# Autodesk Inventor assembly: 14inLift
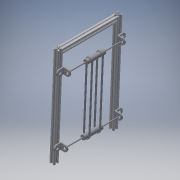
[picture p0: Inventor's stored thumbnail of the model, 180x180]
Saved by Autodesk Inventor 2016 (Build 200138000, 138)
## iProperties
Created: 2016-12-21
Part Number: 14inLift
Document SubType Name: Assembly
Designer: RoboticsUser
Author: RoboticsUser
## Documents named in this file (5)
- C:\Robotics\CAD\2016-17_CAD\12inLift (2).iam
- C:\Robotics\CAD\COTSParts\Bosch Extrusion\Bosch 20x20 16.66 -.ipt
- C:\Robotics\CAD\COTSParts\Actobotics\545 parts\545400_MIR.ipt
- C:\Robotics\CAD\COTSParts\Bosch Extrusion\Bosch 20x20 9 in actual.ipt
- C:\Robotics\CAD\2016-17_CAD\12inlift.iam
## Components (8 placed, 4 different names)
1. Bosch 20x20 16.66 -:1 — Mate:9, Mate:10, Mate:13, Flush:12, Flush:13
2. Bosch 20x20 16.66 -:2 — Mate:11, Mate:12, Mate:14, Flush:16, Flush:17
3. 545400_MIR:1 — Mate:10, Insert:2
4. 545400_MIR:2 — Mate:9, Insert:3
5. 545400_MIR:3 — Mate:11, Insert:1
6. 545400_MIR:4 — Mate:12, Flush:17, Insert:4
7. Bosch 20x20 9 in actual:1 — Mate:13, Flush:12, Flush:13, Mate:14, Flush:16
8. 12inlift:1 [sub-assembly] — Insert:1, Insert:2, Insert:3, Insert:4
## Relationships (14: Mate 6, Flush 4, Insert 4)
- Mate:9: Bosch 20x20 16.66 -:1 ↔ 545400_MIR:2
- Mate:10: Bosch 20x20 16.66 -:1 ↔ 545400_MIR:1
- Mate:11: Bosch 20x20 16.66 -:2 ↔ 545400_MIR:3
- Mate:12: Bosch 20x20 16.66 -:2 ↔ 545400_MIR:4
- Mate:13: Bosch 20x20 16.66 -:1 ↔ Bosch 20x20 9 in actual:1
- Flush:12: Bosch 20x20 16.66 -:1 ↔ Bosch 20x20 9 in actual:1
- Flush:13: Bosch 20x20 16.66 -:1 ↔ Bosch 20x20 9 in actual:1
- Mate:14: Bosch 20x20 16.66 -:2 ↔ Bosch 20x20 9 in actual:1
- Flush:16: Bosch 20x20 16.66 -:2 ↔ Bosch 20x20 9 in actual:1
- Flush:17: Bosch 20x20 16.66 -:2 ↔ 545400_MIR:4
- Insert:1: 545400_MIR:3 ↔ 12inlift:1
- Insert:2: 545400_MIR:1 ↔ 12inlift:1
- Insert:3: 545400_MIR:2 ↔ 12inlift:1
- Insert:4: 545400_MIR:4 ↔ 12inlift:1
